# Autodesk Inventor assembly: solar_harvester_145x145
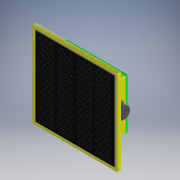
[picture p0: Inventor's stored thumbnail of the model, 180x180]
Saved by Autodesk Inventor 2018 (Build 220112000, 112)
## iProperties
Created: 2019-03-28
Part Number: solar_harvester_145x145
Document SubType Name: Assembly
Designer: ZEUSLAP
Author: ZEUSLAP
## Documents named in this file (12)
- C:\Users\ZEUSLAP\YandexDisk\Inventor\solar_harvester_145x145\solar_harvester_145x145.iam
- C:\Users\ZEUSLAP\YandexDisk\Inventor\solar_harvester_145x145\parts\18650 Battery Holder.ipt
- C:\Users\ZEUSLAP\YandexDisk\Inventor\solar_harvester_145x145\parts\18650 Battery.ipt
- C:\Users\ZEUSLAP\YandexDisk\Inventor\solar_harvester_145x145\parts\Solar Panel 145 x 145 mm.ipt
- C:\Users\ZEUSLAP\YandexDisk\Inventor\solar_harvester_145x145\parts\CN3065 Solar Charger board\CN3065 Solar Charger board.iam
- C:\Users\ZEUSLAP\YandexDisk\Inventor\solar_harvester_145x145\enclosure\solar_panel_back_lid.ipt
- C:\Users\ZEUSLAP\Documents\Inventor\Content Center Files\R2018\en-US\Screw F-Z GOST R ISO 7049-93\Screw ST2.9x9.5-F-Z GOST R ISO 7049-93.ipt
- C:\Users\ZEUSLAP\YandexDisk\Inventor\solar_harvester_145x145\enclosure\solar_board_holder.ipt
- C:\Users\ZEUSLAP\YandexDisk\Inventor\solar_harvester_145x145\enclosure\enclosure_with_bracket.iam
- C:\Users\ZEUSLAP\YandexDisk\Inventor\SP16 waterproof connector\SP16-4P, female, back nut type.iam
- C:\Users\ZEUSLAP\YandexDisk\Inventor\SP16 waterproof connector\parts\nut.ipt
- C:\Users\ZEUSLAP\YandexDisk\Inventor\SP16 waterproof connector\parts\rubber_washer.ipt
## Components (19 placed, 11 different names)
1. 18650 Battery:1 — Mate:5, Mate:6, Angle:2, Angle:5
2. Solar Panel 145 x 145 mm:1 — Mate:7, Mate:14, Mate:15
3. CN3065 Solar Charger board:1 [sub-assembly] — Mate:21, Angle:6, Mate:26, Mate:27
4. solar_panel_back_lid:1 — Mate:16, Mate:17, Mate:18, Mate:19, Angle:5, Mate:20, Mate:21, Angle:6, Mate:24, Mate:25, Mate:26, Mate:27, Rotational:3, Rotational:4, Rotational:5, Rotational:6, Rotational:7, Rotational:8, Mate:34
5. Screw F-Z GOST R ISO 7049-93 ST2.9x9.5:9 — Mate:35, Mate:38
6. solar_board_holder:1 — Mate:24, Mate:25, Mate:34, Mate:35, Mate:36, Mate:37, Mate:38
7. 18650 Battery Holder:1 — Mate:5, Mate:6, Angle:2, Mate:19, Mate:20, Rigid:1
8. enclosure_with_bracket:1 [sub-assembly] — Mate:7, Angle:4, Mate:11, Mate:12, Mate:13, Mate:14, Mate:15, Mate:16, Mate:17, Mate:18, Mate:30, Mate:31, Mate:32
9. Screw F-Z GOST R ISO 7049-93 ST2.9x9.5:10 — Rotational:5
10. Screw F-Z GOST R ISO 7049-93 ST2.9x9.5:11 — Rotational:6
11. Screw F-Z GOST R ISO 7049-93 ST2.9x9.5:12 — Mate:36, Mate:37
12. Screw F-Z GOST R ISO 7049-93 ST2.9x9.5:13 — Rotational:7
13. Screw F-Z GOST R ISO 7049-93 ST2.9x9.5:14 — Rotational:8
14. Screw F-Z GOST R ISO 7049-93 ST2.9x9.5:15 — Rigid:1
15. Screw F-Z GOST R ISO 7049-93 ST2.9x9.5:16 — Rotational:3
16. Screw F-Z GOST R ISO 7049-93 ST2.9x9.5:17 — Rotational:4
17. SP16-4P, female, back nut type:1 [sub-assembly] — Mate:28, Mate:29, Mate:31, Mate:33
18. nut:1 — Mate:32, Mate:33
19. rubber_washer:1 — Mate:28, Mate:29, Mate:30
## Relationships (40: Mate 29, RevoluteJoint 6, Angle 4, WeldJoint 1)
- Mate:5: 18650 Battery:1 ↔ 18650 Battery Holder:1
- Mate:6: 18650 Battery:1 ↔ 18650 Battery Holder:1
- Angle:2 (270 deg): 18650 Battery:1 ↔ 18650 Battery Holder:1
- Mate:7: Solar Panel 145 x 145 mm:1 ↔ enclosure_with_bracket:1
- Angle:4 (0 deg): enclosure_with_bracket:1
- Mate:11: enclosure_with_bracket:1
- Mate:12: enclosure_with_bracket:1
- Mate:13 (85 mm): enclosure_with_bracket:1
- Mate:14 (0.5 mm): Solar Panel 145 x 145 mm:1 ↔ enclosure_with_bracket:1
- Mate:15 (0.5 mm): Solar Panel 145 x 145 mm:1 ↔ enclosure_with_bracket:1
- Mate:16: solar_panel_back_lid:1 ↔ enclosure_with_bracket:1
- Mate:17: solar_panel_back_lid:1 ↔ enclosure_with_bracket:1
- Mate:18: solar_panel_back_lid:1 ↔ enclosure_with_bracket:1
- Mate:19: solar_panel_back_lid:1 ↔ 18650 Battery Holder:1
- Angle:5 (0 deg): 18650 Battery:1 ↔ solar_panel_back_lid:1
- Mate:20: solar_panel_back_lid:1 ↔ 18650 Battery Holder:1
- Mate:21: CN3065 Solar Charger board:1 ↔ solar_panel_back_lid:1
- Angle:6 (180 deg): CN3065 Solar Charger board:1 ↔ solar_panel_back_lid:1
- Mate:24: solar_panel_back_lid:1 ↔ solar_board_holder:1
- Mate:25: solar_panel_back_lid:1 ↔ solar_board_holder:1
- Mate:26 (0.5 mm): CN3065 Solar Charger board:1 ↔ solar_panel_back_lid:1
- Mate:27 (1 mm): CN3065 Solar Charger board:1 ↔ solar_panel_back_lid:1
- Rotational:3 [RevoluteJoint]: solar_panel_back_lid:1 ↔ Screw F-Z GOST R ISO 7049-93 ST2.9x9.5:16
- Rigid:1 [WeldJoint]: 18650 Battery Holder:1 ↔ Screw F-Z GOST R ISO 7049-93 ST2.9x9.5:15
- Rotational:4 [RevoluteJoint]: solar_panel_back_lid:1 ↔ Screw F-Z GOST R ISO 7049-93 ST2.9x9.5:17
- Rotational:5 [RevoluteJoint]: solar_panel_back_lid:1 ↔ Screw F-Z GOST R ISO 7049-93 ST2.9x9.5:10
- Rotational:6 [RevoluteJoint]: solar_panel_back_lid:1 ↔ Screw F-Z GOST R ISO 7049-93 ST2.9x9.5:11
- Rotational:7 [RevoluteJoint]: solar_panel_back_lid:1 ↔ Screw F-Z GOST R ISO 7049-93 ST2.9x9.5:13
- Rotational:8 [RevoluteJoint]: solar_panel_back_lid:1 ↔ Screw F-Z GOST R ISO 7049-93 ST2.9x9.5:14
- Mate:28: SP16-4P, female, back nut type:1 ↔ rubber_washer:1
- Mate:29: SP16-4P, female, back nut type:1 ↔ rubber_washer:1
- Mate:30: enclosure_with_bracket:1 ↔ rubber_washer:1
- Mate:31: enclosure_with_bracket:1 ↔ SP16-4P, female, back nut type:1
- Mate:32: enclosure_with_bracket:1 ↔ nut:1
- Mate:33: SP16-4P, female, back nut type:1 ↔ nut:1
- Mate:34: solar_panel_back_lid:1 ↔ solar_board_holder:1
- Mate:35: Screw F-Z GOST R ISO 7049-93 ST2.9x9.5:9 ↔ solar_board_holder:1
- Mate:36: solar_board_holder:1 ↔ Screw F-Z GOST R ISO 7049-93 ST2.9x9.5:12
- Mate:37: solar_board_holder:1 ↔ Screw F-Z GOST R ISO 7049-93 ST2.9x9.5:12
- Mate:38: Screw F-Z GOST R ISO 7049-93 ST2.9x9.5:9 ↔ solar_board_holder:1
